# Autodesk Inventor assembly: МТ1-3.00.00.00 ЭСБ Сборка
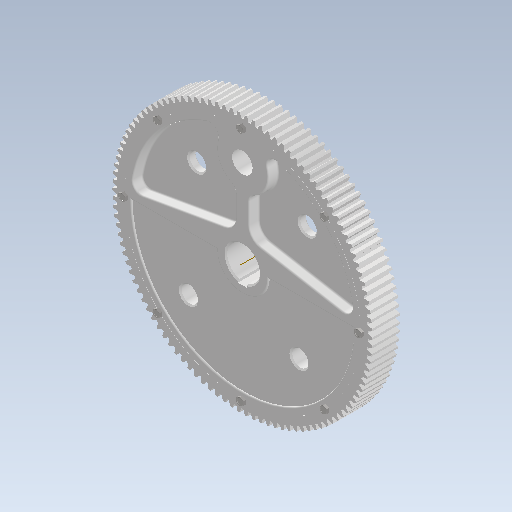
[picture p0: Inventor's stored thumbnail of the model, 512x512]
Saved by Autodesk Inventor 2021 (Build 250183000, 183)
## iProperties
Created: 2022-06-08
Part Number: МТ1-3.00.00.00 ЭСБ Сборка
Document SubType Name: Assembly
Designer: u
Mass: 3316.5 g
Surface Area: 4346.81 cm^2
Volume: 3286.69 cm^3
Density: 1.00907 g/cm^3
Author: u
## Documents named in this file (4)
- C:\Users\u\Documents\Inventor\Projects\AID\МТ1-3.00.00.00 ЭСБ Сборка.iam
- C:\Users\u\Documents\Inventor\Projects\AID\Диск.ipt
- C:\Users\u\Documents\Inventor\Projects\AID\Колесо.ipt
- C:\Users\u\Documents\Inventor\Content Center Files\R2021\ru-RU\Bolt 2 GOST 15591-70\Болт 2 M6×8 ГОСТ 15591-70.ipt
## Components (10 placed, 3 different names)
1. Диск:1 — Заподлицо:1, Заподлицо:2, Заподлицо:3, Совмещение:1, Заподлицо:4, Вставка:1, Вставка:2, Вставка:3, Вставка:4, Вставка:5, Вставка:6, Вставка:7, Вставка:8
2. Колесо:1 — Совмещение:1, Заподлицо:4, Заподлицо:5
3. Болт 2 ГОСТ 15591-70 M6×8:1 — Вставка:1
4. Болт 2 ГОСТ 15591-70 M6×8:2 — Вставка:2
5. Болт 2 ГОСТ 15591-70 M6×8:3 — Вставка:3
6. Болт 2 ГОСТ 15591-70 M6×8:4 — Вставка:4
7. Болт 2 ГОСТ 15591-70 M6×8:5 — Вставка:5
8. Болт 2 ГОСТ 15591-70 M6×8:6 — Вставка:6
9. Болт 2 ГОСТ 15591-70 M6×8:7 — Вставка:7
10. Болт 2 ГОСТ 15591-70 M6×8:8 — Вставка:8
## Relationships (14: Insert 8, Flush 5, Mate 1)
- Заподлицо:1 [Flush]: Диск:1
- Заподлицо:2 [Flush]: Диск:1
- Заподлицо:3 [Flush]: Диск:1
- Совмещение:1 [Mate]: Диск:1 ↔ Колесо:1
- Заподлицо:4 [Flush]: Диск:1 ↔ Колесо:1
- Заподлицо:5 [Flush]: Колесо:1
- Вставка:1 [Insert]: Диск:1 ↔ Болт 2 ГОСТ 15591-70 M6×8:1
- Вставка:2 [Insert]: Диск:1 ↔ Болт 2 ГОСТ 15591-70 M6×8:2
- Вставка:3 [Insert]: Диск:1 ↔ Болт 2 ГОСТ 15591-70 M6×8:3
- Вставка:4 [Insert]: Диск:1 ↔ Болт 2 ГОСТ 15591-70 M6×8:4
- Вставка:5 [Insert]: Диск:1 ↔ Болт 2 ГОСТ 15591-70 M6×8:5
- Вставка:6 [Insert]: Диск:1 ↔ Болт 2 ГОСТ 15591-70 M6×8:6
- Вставка:7 [Insert]: Диск:1 ↔ Болт 2 ГОСТ 15591-70 M6×8:7
- Вставка:8 [Insert]: Диск:1 ↔ Болт 2 ГОСТ 15591-70 M6×8:8
